# Autodesk Inventor assembly: 1_Body_Cam1
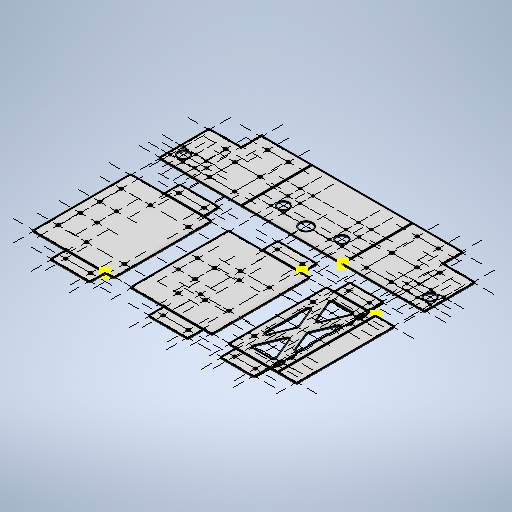
[picture p0: Inventor's stored thumbnail of the model, 512x512]
Saved by Autodesk Inventor 2026.1 (Build 301233000, 233)
## iProperties
Created: 2025-08-16
Part Number: 1_Body_Cam1
Document SubType Name: Assembly
Designer: chris
Author: chris
## Documents named in this file (5)
- C:\Users\chris\Documents\Inventor\RHp_Humanoid_ver1\Cam\Body\1.5T\Assembly\1_Body_Cam1.iam
- C:\Users\chris\Documents\Inventor\RHp_Humanoid_ver1\Cam\Body\1.5T\Part\body_main_frame.ipt
- C:\Users\chris\Documents\Inventor\RHp_Humanoid_ver1\Cam\Body\1.5T\Part\body_front_frame.ipt
- C:\Users\chris\Documents\Inventor\RHp_Humanoid_ver1\Cam\Body\1.5T\Part\body_middle_frame.ipt
- C:\Users\chris\Documents\Inventor\RHp_Humanoid_ver1\Cam\Body\1.5T\Part\body_back_frame.ipt
## Components (4 placed, 4 different names)
1. body_main_frame:1 — Mate:1, Mate:2, Flush:1, Flush:2, Flush:4, Mate:3, Mate:5, Flush:5, Flush:6, Mate:6
2. body_front_frame:1 — Flush:2, Mate:3, Flush:5, Mate:7
3. body_back_frame:1 — Flush:4, Mate:5, Mate:8
4. body_middle_frame:1 — Flush:6, Mate:6, Mate:7, Mate:8
## Relationships (12: Mate 7, Flush 5)
- Mate:1: body_main_frame:1
- Mate:2: body_main_frame:1
- Flush:1: body_main_frame:1
- Flush:2: body_main_frame:1 ↔ body_front_frame:1
- Flush:4: body_main_frame:1 ↔ body_back_frame:1
- Mate:3 (15 mm): body_main_frame:1 ↔ body_front_frame:1
- Mate:5 (15 mm): body_main_frame:1 ↔ body_back_frame:1
- Flush:5: body_main_frame:1 ↔ body_front_frame:1
- Flush:6: body_main_frame:1 ↔ body_middle_frame:1
- Mate:6 (15 mm): body_main_frame:1 ↔ body_middle_frame:1
- Mate:7 (20 mm): body_front_frame:1 ↔ body_middle_frame:1
- Mate:8 (20 mm): body_back_frame:1 ↔ body_middle_frame:1
